# Autodesk Inventor assembly: 組合1
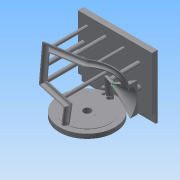
[picture p0: Inventor's stored thumbnail of the model, 180x180]
Saved by Autodesk Inventor 2015 (Build 190159000, 159)
## iProperties
Created: 2018-04-17
Part Number: 組合1
Document SubType Name: Assembly
Designer: 王博聖
Author: 王博聖
## Documents named in this file (6)
- C:\Users\王博聖\Desktop\FF\組合1.iam
- C:\Users\王博聖\Desktop\FF\零件1.ipt
- C:\Users\王博聖\Desktop\FF\零件2.ipt
- C:\Users\王博聖\Desktop\FF\零件3.ipt
- C:\Users\王博聖\Desktop\FF\零件4.ipt
- C:\Users\王博聖\Desktop\FF\零件5.ipt
## Components (5 placed, 5 different names)
1. 零件1:1 — 貼合:1, 貼合:2, 貼合:3, 貼合:4, 貼合:5
2. 零件2:1 — 貼合:3, 貼合:4, 貼合:5, 齊平:1, 齊平:2
3. 零件3:1 — 貼合:1, 貼合:2, 齊平:3, 齊平:4, 貼合:6
4. 零件4:1 — 齊平:1, 齊平:2, 齊平:3, 齊平:4
5. 零件5:1 — 貼合:6
## Relationships (10: Mate 6, Flush 4)
- 貼合:1 [Mate]: 零件1:1 ↔ 零件3:1
- 貼合:2 [Mate]: 零件1:1 ↔ 零件3:1
- 貼合:3 [Mate]: 零件1:1 ↔ 零件2:1
- 貼合:4 [Mate]: 零件1:1 ↔ 零件2:1
- 貼合:5 [Mate]: 零件1:1 ↔ 零件2:1
- 齊平:1 [Flush]: 零件2:1 ↔ 零件4:1
- 齊平:2 [Flush]: 零件2:1 ↔ 零件4:1
- 齊平:3 [Flush] (-95 mm): 零件3:1 ↔ 零件4:1
- 齊平:4 [Flush]: 零件3:1 ↔ 零件4:1
- 貼合:6 [Mate]: 零件3:1 ↔ 零件5:1
